# Autodesk Inventor assembly: AS-00000000
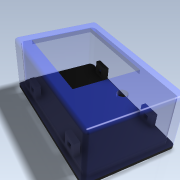
[picture p0: Inventor's stored thumbnail of the model, 180x180]
Saved by Autodesk Inventor 2020.1 (Build 241239000, 239)
## iProperties
Company: Haynie Research & Development, LLC
Created: 2020-09-08
Part Number: AS-00000000
Document SubType Name: Assembly
Designer: Lance Haynie
Engineer: Lance Haynie
Author: Haynie R&D
## Documents named in this file (3)
- C:\Users\hrd\Documents\Vault\Haynie Research\Telemetry\Receiver Box\Receiver Box.iam
- C:\Users\hrd\Documents\Vault\Haynie Research\Telemetry\Receiver Box\receiver-box.ipt
- C:\Users\hrd\Documents\Vault\Haynie Research\Telemetry\Receiver Box\receiver-box-lid.ipt
## Components (2 placed, 2 different names)
1. receiver-box:1 — Mate:1, Mate:2, Mate:3
2. receiver-box-lid:1 — Mate:1, Mate:2, Mate:3
## Relationships (3: Mate 3)
- Mate:1: receiver-box:1 ↔ receiver-box-lid:1
- Mate:2: receiver-box:1 ↔ receiver-box-lid:1
- Mate:3: receiver-box:1 ↔ receiver-box-lid:1
